# Autodesk Inventor assembly: Griber samlet
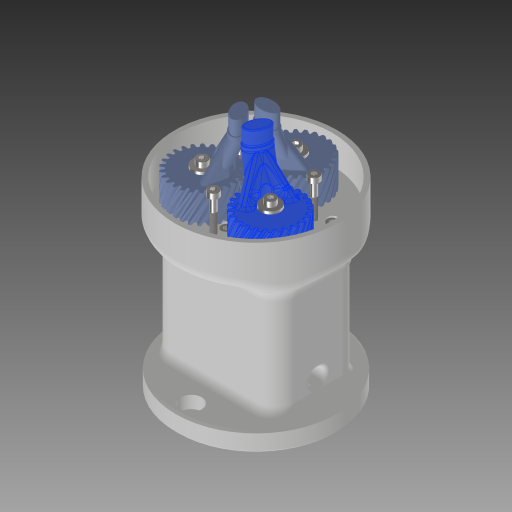
[picture p0: Inventor's stored thumbnail of the model, 512x512]
Saved by Autodesk Inventor 2024 (Build 280153000, 153)
## iProperties
Created: 2024-03-08
Part Number: Griber samlet
Document SubType Name: Assembly
Designer: Faber
Author: Faber
## Documents named in this file (11)
- C:\Users\Bluex\Documents\GitHub\Autonome_Robotter\3D_inventor_robor_hånd\Griber samlet_V1b.iam
- C:\Users\Bluex\OneDrive - Syddansk Universitet\2. Semester\Semesterprojekt i autonome robotter\Inventor filer\Sol_Gear.ipt
- C:\Users\Bluex\OneDrive - Syddansk Universitet\2. Semester\Semesterprojekt i autonome robotter\Inventor filer\Gear_Hus_V1b.ipt
- C:\Users\Bluex\OneDrive - Syddansk Universitet\2. Semester\Semesterprojekt i autonome robotter\Inventor filer\Gear_Hus_Laag_V1b.ipt
- C:\Users\Bluex\OneDrive - Syddansk Universitet\2. Semester\Semesterprojekt i autonome robotter\Inventor filer\Motor_Hus_V1b.ipt
- C:\Users\Bluex\Documents\Inventor\Content Center Files\R2024\en-US\ISO 4032(1)\ISO 4032 - M3DIN EN.ipt
- C:\Users\Bluex\Documents\Inventor\Content Center Files\R2024\en-US\ISO 4762(1)\DIN EN ISO 4762 - M3 x 16.ipt
- C:\Users\Bluex\Documents\Inventor\Content Center Files\R2024\en-US\ISO 4762(1)\DIN EN ISO 4762 - M3 x 8.ipt
- C:\Users\Bluex\Documents\Inventor\Content Center Files\R2024\en-US\ISO 4762(1)\DIN EN ISO 4762 - M3 x 25.ipt
- C:\Users\Bluex\Documents\GitHub\Autonome_Robotter\3D_inventor_robor_hånd\Planet_Gear_finger_V2b.ipt
- C:\Users\Bluex\Documents\Inventor\Content Center Files\R2024\en-US\ANSI B18.22 M\ANSI B18.22M - 3.5 R.ipt
## Components (30 placed, 10 different names)
1. Sol_Gear:1 — Mate:2, Mate:3, Rotation:4, Rotation:5, Rotation:6
2. Gear_Hus_V1b:1 — Mate:2, Mate:3, Mate:4, Mate:5, Mate:6, Mate:7, Mate:8, Mate:9, Mate:24, Mate:25, Mate:26, Mate:27, Mate:28, Mate:29, Mate:30, Mate:31, Mate:32, Mate:33, Mate:34, Mate:35, Mate:36, Mate:37, Mate:38, Mate:39, Mate:40, Mate:41, Mate:42, Mate:43, Mate:50, Mate:51, Mate:52, Mate:53, Mate:54, Mate:55, Mate:56, Mate:57, Mate:58, Mate:59, Mate:61, Mate:63
3. Gear_Hus_Laag_V1b:1 — Mate:4, Mate:5, Mate:6, Mate:44, Mate:45, Mate:46, Mate:47, Mate:48, Mate:49
4. Motor_Hus_V1b:1 — Mate:7, Mate:8, Mate:9, Mate:16, Mate:17, Mate:18, Mate:19, Mate:20, Mate:21, Mate:22, Mate:23
5. DIN EN 24032 M3:1 — Mate:16, Mate:17
6. DIN EN 24032 M3:2 — Mate:18, Mate:19
7. DIN EN 24032 M3:3 — Mate:20, Mate:21
8. DIN EN 24032 M3:4 — Mate:22, Mate:23
9. DIN EN ISO 4762 M3 x 16:1 — Mate:24, Mate:25
10. DIN EN ISO 4762 M3 x 16:2 — Mate:30, Mate:35
11. DIN EN ISO 4762 M3 x 16:3 — Mate:26, Mate:34
12. DIN EN ISO 4762 M3 x 16:4 — Mate:31, Mate:33
13. DIN EN ISO 4762 M3 x 8:1 — Mate:27, Mate:37
14. DIN EN ISO 4762 M3 x 8:2 — Mate:29, Mate:36
15. DIN EN ISO 4762 M3 x 8:3 — Mate:28, Mate:32
16. DIN EN 24032 M3:5 — Mate:38, Mate:43
17. DIN EN 24032 M3:6 — Mate:39, Mate:40
18. DIN EN 24032 M3:7 — Mate:41, Mate:42
19. DIN EN ISO 4762 M3 x 25:1 — Mate:44, Mate:45
20. DIN EN ISO 4762 M3 x 25:2 — Mate:46, Mate:49
21. DIN EN ISO 4762 M3 x 25:3 — Mate:47, Mate:48
22. DIN EN ISO 4762 M3 x 8:4 — Mate:50, Mate:64, Mate:66
23. DIN EN ISO 4762 M3 x 8:5 — Mate:51, Mate:60, Mate:67
24. DIN EN ISO 4762 M3 x 8:6 — Mate:52, Mate:62, Mate:65
25. Planet_Gear_finger_V2b:1 — Mate:53, Mate:54, Rotation:4
26. Planet_Gear_finger_V2b:2 — Mate:55, Mate:56, Rotation:6
27. Planet_Gear_finger_V2b:3 — Mate:57, Mate:58, Rotation:5
28. Plain Washer (Metric) 3.5 R:1 — Mate:63, Mate:64, Mate:66
29. Plain Washer (Metric) 3.5 R:2 — Mate:61, Mate:62, Mate:65
30. Plain Washer (Metric) 3.5 R:3 — Mate:59, Mate:60, Mate:67
## Relationships (63: Mate 60, RelateRotation 3)
- Mate:2: Sol_Gear:1 ↔ Gear_Hus_V1b:1
- Mate:3: Sol_Gear:1 ↔ Gear_Hus_V1b:1
- Mate:4: Gear_Hus_V1b:1 ↔ Gear_Hus_Laag_V1b:1
- Mate:5: Gear_Hus_V1b:1 ↔ Gear_Hus_Laag_V1b:1
- Mate:6: Gear_Hus_V1b:1 ↔ Gear_Hus_Laag_V1b:1
- Mate:7: Gear_Hus_V1b:1 ↔ Motor_Hus_V1b:1
- Mate:8: Gear_Hus_V1b:1 ↔ Motor_Hus_V1b:1
- Mate:9: Gear_Hus_V1b:1 ↔ Motor_Hus_V1b:1
- Mate:16: Motor_Hus_V1b:1 ↔ DIN EN 24032 M3:1
- Mate:17: Motor_Hus_V1b:1 ↔ DIN EN 24032 M3:1
- Mate:18: Motor_Hus_V1b:1 ↔ DIN EN 24032 M3:2
- Mate:19: Motor_Hus_V1b:1 ↔ DIN EN 24032 M3:2
- Mate:20: Motor_Hus_V1b:1 ↔ DIN EN 24032 M3:3
- Mate:21: Motor_Hus_V1b:1 ↔ DIN EN 24032 M3:3
- Mate:22: Motor_Hus_V1b:1 ↔ DIN EN 24032 M3:4
- Mate:23: Motor_Hus_V1b:1 ↔ DIN EN 24032 M3:4
- Mate:24: Gear_Hus_V1b:1 ↔ DIN EN ISO 4762 M3 x 16:1
- Mate:25: Gear_Hus_V1b:1 ↔ DIN EN ISO 4762 M3 x 16:1
- Mate:26: Gear_Hus_V1b:1 ↔ DIN EN ISO 4762 M3 x 16:3
- Mate:27: Gear_Hus_V1b:1 ↔ DIN EN ISO 4762 M3 x 8:1
- Mate:28: Gear_Hus_V1b:1 ↔ DIN EN ISO 4762 M3 x 8:3
- Mate:29: Gear_Hus_V1b:1 ↔ DIN EN ISO 4762 M3 x 8:2
- Mate:30: Gear_Hus_V1b:1 ↔ DIN EN ISO 4762 M3 x 16:2
- Mate:31: Gear_Hus_V1b:1 ↔ DIN EN ISO 4762 M3 x 16:4
- Mate:32: Gear_Hus_V1b:1 ↔ DIN EN ISO 4762 M3 x 8:3
- Mate:33: Gear_Hus_V1b:1 ↔ DIN EN ISO 4762 M3 x 16:4
- Mate:34: Gear_Hus_V1b:1 ↔ DIN EN ISO 4762 M3 x 16:3
- Mate:35: Gear_Hus_V1b:1 ↔ DIN EN ISO 4762 M3 x 16:2
- Mate:36: Gear_Hus_V1b:1 ↔ DIN EN ISO 4762 M3 x 8:2
- Mate:37: Gear_Hus_V1b:1 ↔ DIN EN ISO 4762 M3 x 8:1
- Mate:38: Gear_Hus_V1b:1 ↔ DIN EN 24032 M3:5
- Mate:39: Gear_Hus_V1b:1 ↔ DIN EN 24032 M3:6
- Mate:40: Gear_Hus_V1b:1 ↔ DIN EN 24032 M3:6
- Mate:41: Gear_Hus_V1b:1 ↔ DIN EN 24032 M3:7
- Mate:42: Gear_Hus_V1b:1 ↔ DIN EN 24032 M3:7
- Mate:43: Gear_Hus_V1b:1 ↔ DIN EN 24032 M3:5
- Mate:44: Gear_Hus_Laag_V1b:1 ↔ DIN EN ISO 4762 M3 x 25:1
- Mate:45: Gear_Hus_Laag_V1b:1 ↔ DIN EN ISO 4762 M3 x 25:1
- Mate:46: Gear_Hus_Laag_V1b:1 ↔ DIN EN ISO 4762 M3 x 25:2
- Mate:47: Gear_Hus_Laag_V1b:1 ↔ DIN EN ISO 4762 M3 x 25:3
- Mate:48: Gear_Hus_Laag_V1b:1 ↔ DIN EN ISO 4762 M3 x 25:3
- Mate:49: Gear_Hus_Laag_V1b:1 ↔ DIN EN ISO 4762 M3 x 25:2
- Mate:50: Gear_Hus_V1b:1 ↔ DIN EN ISO 4762 M3 x 8:4
- Mate:51: Gear_Hus_V1b:1 ↔ DIN EN ISO 4762 M3 x 8:5
- Mate:52: Gear_Hus_V1b:1 ↔ DIN EN ISO 4762 M3 x 8:6
- Mate:53: Gear_Hus_V1b:1 ↔ Planet_Gear_finger_V2b:1
- Mate:54: Gear_Hus_V1b:1 ↔ Planet_Gear_finger_V2b:1
- Rotation:4 [RelateRotation] (0.3846 ul): Sol_Gear:1 ↔ Planet_Gear_finger_V2b:1
- Mate:55: Gear_Hus_V1b:1 ↔ Planet_Gear_finger_V2b:2
- Mate:56: Gear_Hus_V1b:1 ↔ Planet_Gear_finger_V2b:2
- Mate:57: Gear_Hus_V1b:1 ↔ Planet_Gear_finger_V2b:3
- Mate:58: Gear_Hus_V1b:1 ↔ Planet_Gear_finger_V2b:3
- Mate:59: Gear_Hus_V1b:1 ↔ Plain Washer (Metric) 3.5 R:3
- Mate:60: DIN EN ISO 4762 M3 x 8:5 ↔ Plain Washer (Metric) 3.5 R:3
- Mate:61: Gear_Hus_V1b:1 ↔ Plain Washer (Metric) 3.5 R:2
- Mate:62: DIN EN ISO 4762 M3 x 8:6 ↔ Plain Washer (Metric) 3.5 R:2
- Mate:63: Gear_Hus_V1b:1 ↔ Plain Washer (Metric) 3.5 R:1
- Mate:64: DIN EN ISO 4762 M3 x 8:4 ↔ Plain Washer (Metric) 3.5 R:1
- Rotation:5 [RelateRotation] (0.3846 ul): Sol_Gear:1 ↔ Planet_Gear_finger_V2b:3
- Rotation:6 [RelateRotation] (0.3846 ul): Sol_Gear:1 ↔ Planet_Gear_finger_V2b:2
- Mate:65: DIN EN ISO 4762 M3 x 8:6 ↔ Plain Washer (Metric) 3.5 R:2
- Mate:66: DIN EN ISO 4762 M3 x 8:4 ↔ Plain Washer (Metric) 3.5 R:1
- Mate:67: DIN EN ISO 4762 M3 x 8:5 ↔ Plain Washer (Metric) 3.5 R:3
## Named parameters: Finish4_Area = 0.118936
note: some values were not read from the file. Shown as the stored number, unit unknown: "Finish4_Area".
